# Autodesk Inventor assembly: Aktutator
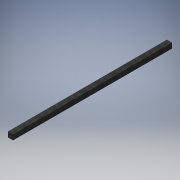
[picture p0: Inventor's stored thumbnail of the model, 180x180]
Saved by Autodesk Inventor 2017 (Build 210142000, 142)
## iProperties
Created: 2016-07-21
Part Number: Aktutator
Document SubType Name: Assembly
Designer: Marcin
Mass: 37524.2 g
Surface Area: 5308.39 cm^2
Volume: 4780.15 cm^3
Density: 7.85 g/cm^3
Author: Marcin
## Documents named in this file (3)
- M:\PracaInżynierska\Aktutator.iam
- M:\PracaInżynierska\Cylinder.ipt
- M:\PracaInżynierska\tlok.ipt
## Components (2 placed, 2 different names)
1. Cylinder:1 — Cylindrical:1
2. tlok:1 — Cylindrical:1
## Relationships (1: CylindricalJoint 1)
- Cylindrical:1: Cylinder:1 ↔ tlok:1
